# Autodesk Inventor assembly: robot
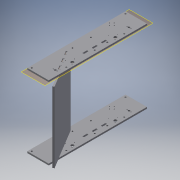
[picture p0: Inventor's stored thumbnail of the model, 180x180]
Saved by Autodesk Inventor 2019 (Build 230136000, 136)
## iProperties
Created: 2019-11-04
Part Number: robot
Document SubType Name: Assembly
Designer: shrey
Author: shrey
## Documents named in this file (3)
- C:\Users\shrey\Desktop\4326Cad\robot.iam
- C:\Users\shrey\Desktop\4326Cad\ChassisInsideWithFlower.ipt
- C:\Users\shrey\Desktop\4326Cad\ramp.ipt
## Components (3 placed, 2 different names)
1. ChassisInsideWithFlower:1 — Flush:1, Mate:1, Mate:2, Rigid:1
2. ChassisInsideWithFlower:2 — Flush:1, Mate:1, Flush:2
3. ramp:1 — Rigid:1
## Relationships (5: Flush 2, Mate 2, WeldJoint 1)
- Flush:1: ChassisInsideWithFlower:1 ↔ ChassisInsideWithFlower:2
- Mate:1: ChassisInsideWithFlower:1 ↔ ChassisInsideWithFlower:2
- Flush:2 (292.1 mm): ChassisInsideWithFlower:2
- Mate:2: ChassisInsideWithFlower:1
- Rigid:1 [WeldJoint]: ChassisInsideWithFlower:1 ↔ ramp:1
